# Autodesk Inventor assembly: Unit_MR-O
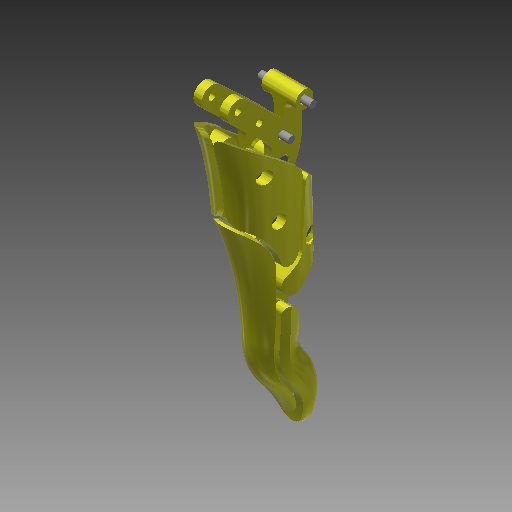
[picture p0: Inventor's stored thumbnail of the model, 512x512]
Saved by Autodesk Inventor 2018.2 (Build 222227000, 227)
## iProperties
Created: 2017-09-22
Part Number: Unit_MR-O
Material: 一般
Document SubType Name: Assembly
Designer: sktom
Author: sktom
Title: Unit_MR-O
## Documents named in this file (9)
- D:\CloudStrage\OneDrive\CADMech\HbSizeMMech\UnitHand\Unit_MR-H\Unit_MR-O\Unit_MR-O.iam
- D:\CloudStrage\OneDrive\CADMech\HbSizeMMech\UnitHand\Unit_MR-H\Unit_MR-O\Dummy_JointPosition.ipt
- D:\CloudStrage\OneDrive\CADMech\HbSizeMMech\UnitHand\Unit_MR-H\Unit_MR-O\MR-O-01.ipt
- D:\CloudStrage\OneDrive\CADMech\HbSizeMMech\UnitHand\Unit_MR-H\Unit_MR-O\MR-O-02.ipt
- D:\CloudStrage\OneDrive\CADMech\HbSizeMMech\UnitHand\Unit_MR-H\Unit_MR-O\MR-O-03.ipt
- D:\CloudStrage\OneDrive\CADMech\HbSizeMMech\UnitHand\Unit_MR-H\Unit_MR-O\MR-O-04.ipt
- D:\CloudStrage\OneDrive\CADMech\HbSizeMMech\UnitHand\Unit_MR-H\Unit_MR-O\MR-O-05.ipt
- D:\CloudStrage\OneDrive\CADMech\HbSizeMMech\UnitHand\Unit_MR-H\Unit_MR-O\Parts_Shaft_Phi2_L8.ipt
- D:\CloudStrage\OneDrive\CADMech\HbSizeMMech\UnitHand\Unit_MR-H\Unit_MR-O\Parts_Screw_M1.7_L8.ipt
## Components (12 placed, 8 different names)
1. Dummy_Position — 回転:4, 回転:6, 回転:7, 円柱状:8
2. MR-O-01 — 回転:5, 円柱状:5, 円柱状:6, 円柱状:7, メイト:1
3. MR-O-02 — 回転:7, 円柱状:6, 挿入:7, 挿入:8
4. MR-O-03 — 円柱状:7, 円柱状:8, 挿入:5, 挿入:6, メイト:1
5. MR-O-04 — 挿入:1, 挿入:2, 挿入:5, 挿入:6
6. MR-O-05 — 挿入:3, 挿入:4, 挿入:7, 挿入:8
7. Parts_Screw_M1.7_L8:1 — 挿入:1
8. Parts_Screw_M1.7_L8:2 — 挿入:2
9. Parts_Screw_M1.7_L8:3 — 挿入:3
10. Parts_Screw_M1.7_L8:4 — 挿入:4
11. Parts_Shaft_Phi2_L8:1 — 回転:4, 回転:5
12. Parts_Shaft_Phi2_L8:2 — 回転:6, 円柱状:5
## Relationships (17: Insert 8, RevoluteJoint 4, CylindricalJoint 4, Mate 1)
- 挿入:1 [Insert]: MR-O-04 ↔ Parts_Screw_M1.7_L8:1
- 挿入:2 [Insert]: MR-O-04 ↔ Parts_Screw_M1.7_L8:2
- 挿入:3 [Insert]: MR-O-05 ↔ Parts_Screw_M1.7_L8:3
- 挿入:4 [Insert]: MR-O-05 ↔ Parts_Screw_M1.7_L8:4
- 回転:4 [RevoluteJoint]: Dummy_Position ↔ Parts_Shaft_Phi2_L8:1
- 回転:6 [RevoluteJoint]: Dummy_Position ↔ Parts_Shaft_Phi2_L8:2
- 回転:5 [RevoluteJoint]: MR-O-01 ↔ Parts_Shaft_Phi2_L8:1
- 円柱状:5 [CylindricalJoint]: MR-O-01 ↔ Parts_Shaft_Phi2_L8:2
- 回転:7 [RevoluteJoint]: Dummy_Position ↔ MR-O-02
- 円柱状:6 [CylindricalJoint]: MR-O-01 ↔ MR-O-02
- 円柱状:7 [CylindricalJoint]: MR-O-01 ↔ MR-O-03
- 円柱状:8 [CylindricalJoint]: Dummy_Position ↔ MR-O-03
- 挿入:5 [Insert]: MR-O-03 ↔ MR-O-04
- 挿入:6 [Insert]: MR-O-03 ↔ MR-O-04
- 挿入:7 [Insert]: MR-O-02 ↔ MR-O-05
- 挿入:8 [Insert]: MR-O-02 ↔ MR-O-05
- メイト:1 [Mate] (0.35 mm): MR-O-01 ↔ MR-O-03
